# Autodesk Inventor assembly: MCI_PCB
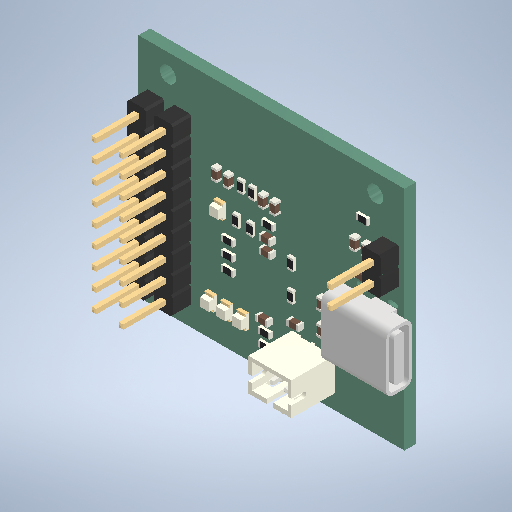
[picture p0: Inventor's stored thumbnail of the model, 512x512]
Saved by Autodesk Inventor 2025.2 (Build 292293000, 293)
## iProperties
Company: Kicad
Created: 2024-11-11
Part Number: MCI_PCB
Description: KiCad electronic assembly
Document SubType Name: Assembly
Designer: matss
Authority: Unknown
Sending System: KiCad to STEP converter
Preprocessor: Open CASCADE STEP processor 7.8
Title: MCI_PCB.step
Author: Pcbnew
## Documents named in this file (10)
- C:\Users\matss\Documents\.Studium\Health_Device\CAD\Wearable-Health-Device\MCI_PCB\MCI_PCB\MCI_PCB.iam
- C:\Users\matss\Documents\.Studium\Health_Device\CAD\Wearable-Health-Device\MCI_PCB\MCI_PCB\R_0603_1608Metric.iam
- C:\Users\matss\Documents\.Studium\Health_Device\CAD\Wearable-Health-Device\MCI_PCB\MCI_PCB\C_0603_1608Metric.iam
- C:\Users\matss\Documents\.Studium\Health_Device\CAD\Wearable-Health-Device\MCI_PCB\MCI_PCB\PinHeader_1x09_P2.54mm_Vertical.iam
- C:\Users\matss\Documents\.Studium\Health_Device\CAD\Wearable-Health-Device\MCI_PCB\MCI_PCB\LED_0805_2012Metric.iam
- C:\Users\matss\Documents\.Studium\Health_Device\CAD\Wearable-Health-Device\MCI_PCB\MCI_PCB\USON-10_2.5x1.0mm_P0.5mm.iam
- C:\Users\matss\Documents\.Studium\Health_Device\CAD\Wearable-Health-Device\MCI_PCB\MCI_PCB\JST_PH_B2B-PH-K_1x02_P2.00mm_Vertical.iam
- C:\Users\matss\Documents\.Studium\Health_Device\CAD\Wearable-Health-Device\MCI_PCB\MCI_PCB\PinHeader_1x02_P2.54mm_Vertical.iam
- C:\Users\matss\Documents\.Studium\Health_Device\CAD\Wearable-Health-Device\MCI_PCB\MCI_PCB\MCI_PCB_PCB.ipt
- C:\Users\matss\Documents\.Studium\Health_Device\CAD\Wearable-Health-Device\USB-C.ipt
## Components (41 placed, 41 different names)
1. 2 [sub-assembly]
2. 4 [sub-assembly]
3. 6 [sub-assembly]
4. 7 [sub-assembly]
5. 8 [sub-assembly]
6. 10 [sub-assembly]
7. 11 [sub-assembly]
8. 12 [sub-assembly]
9. 14 [sub-assembly]
10. 15 [sub-assembly]
11. 16 [sub-assembly]
12. 17 [sub-assembly]
13. 18 [sub-assembly]
14. 19 [sub-assembly]
15. 20 [sub-assembly]
16. 21 [sub-assembly]
17. 22 [sub-assembly]
18. 23 [sub-assembly]
19. 24 [sub-assembly]
20. 26 [sub-assembly]
21. 27 [sub-assembly]
22. 28 [sub-assembly]
23. 29 [sub-assembly]
24. 30 [sub-assembly]
25. 32 [sub-assembly]
26. 33 [sub-assembly]
27. 34 [sub-assembly]
28. 35 [sub-assembly]
29. 36 [sub-assembly]
30. 37 [sub-assembly]
31. 38 [sub-assembly]
32. 39 [sub-assembly]
33. 40 [sub-assembly]
34. 41 [sub-assembly]
35. 42 [sub-assembly]
36. 43 [sub-assembly]
37. 44 [sub-assembly]
38. 45 [sub-assembly]
39. 46 [sub-assembly]
40. 47 — Mate:1, Flush:1, Flush:2
41. USB-C:1 — Mate:1, Flush:1, Flush:2
## Relationships (3: Flush 2, Mate 1)
- Mate:1: 47 ↔ USB-C:1
- Flush:1: 47 ↔ USB-C:1
- Flush:2 (-1 mm): 47 ↔ USB-C:1
